# Autodesk Inventor assembly: main
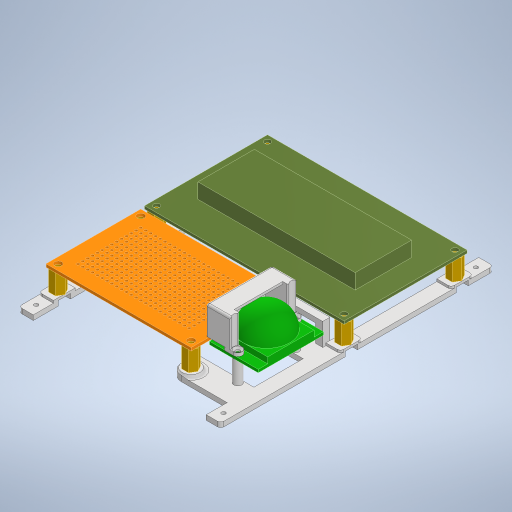
[picture p0: Inventor's stored thumbnail of the model, 512x512]
Saved by Autodesk Inventor 2023 (Build 270158000, 158)
## iProperties
Created: 2023-04-16
Part Number: main
Document SubType Name: Assembly
Designer: taka2
Author: taka2
## Documents named in this file (8)
- C:\Users\taka2\OneDrive\ドキュメント\04Myproject\Modeling\Inventor\clock_room\main.iam
- C:\Users\taka2\OneDrive\ドキュメント\04Myproject\Modeling\Inventor\clock_room\base.ipt
- C:\Users\taka2\OneDrive\ドキュメント\04Myproject\Modeling\Inventor\clock_room\sensorjoint.ipt
- C:\Users\taka2\OneDrive\ドキュメント\04Myproject\Modeling\Inventor\template\LCD_module.ipt
- C:\Users\taka2\OneDrive\ドキュメント\04Myproject\Modeling\Inventor\template\ユニバーサル基盤_ICB-88.ipt
- C:\Users\taka2\OneDrive\ドキュメント\04Myproject\Modeling\Inventor\template\スペーサー_10mm.ipt
- C:\Users\taka2\OneDrive\ドキュメント\04Myproject\Modeling\Inventor\template\人感センサモジュール.ipt
- C:\Users\taka2\OneDrive\ドキュメント\04Myproject\Modeling\Inventor\clock_room\sensorcover.ipt
## Components (15 placed, 7 different names)
1. base:1 — リジッド:1, リジッド:2, リジッド:3, リジッド:4, リジッド:5, リジッド:6, リジッド:7, リジッド:8, リジッド:10, リジッド:9
2. sensorjoint:1 — リジッド:1, リジッド:14
3. sensorjoint:2 — リジッド:2
4. スペーサー_10mm:1 — リジッド:3
5. スペーサー_10mm:2 — リジッド:5
6. スペーサー_10mm:3 — リジッド:6, リジッド:11
7. スペーサー_10mm:4 — リジッド:8
8. スペーサー_10mm:5 — リジッド:9
9. スペーサー_10mm:6 — リジッド:10, リジッド:13
10. スペーサー_10mm:7 — リジッド:7
11. スペーサー_10mm:8 — リジッド:4
12. LCD_module:1 — リジッド:11
13. ユニバーサル基盤_ICB-88:1 — リジッド:13
14. 人感センサモジュール:1 — リジッド:14, リジッド:15
15. sensorcover:1 — リジッド:15
## Relationships (14: WeldJoint 14)
- リジッド:1 [WeldJoint]: base:1 ↔ sensorjoint:1
- リジッド:2 [WeldJoint]: base:1 ↔ sensorjoint:2
- リジッド:3 [WeldJoint]: base:1 ↔ スペーサー_10mm:1
- リジッド:4 [WeldJoint]: base:1 ↔ スペーサー_10mm:8
- リジッド:5 [WeldJoint]: base:1 ↔ スペーサー_10mm:2
- リジッド:6 [WeldJoint]: base:1 ↔ スペーサー_10mm:3
- リジッド:7 [WeldJoint]: base:1 ↔ スペーサー_10mm:7
- リジッド:8 [WeldJoint]: base:1 ↔ スペーサー_10mm:4
- リジッド:10 [WeldJoint]: base:1 ↔ スペーサー_10mm:6
- リジッド:9 [WeldJoint]: base:1 ↔ スペーサー_10mm:5
- リジッド:13 [WeldJoint]: スペーサー_10mm:6 ↔ ユニバーサル基盤_ICB-88:1
- リジッド:11 [WeldJoint]: スペーサー_10mm:3 ↔ LCD_module:1
- リジッド:14 [WeldJoint]: sensorjoint:1 ↔ 人感センサモジュール:1
- リジッド:15 [WeldJoint]: 人感センサモジュール:1 ↔ sensorcover:1
